# Autodesk Inventor assembly: inner_guide_asm
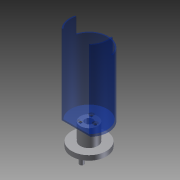
[picture p0: Inventor's stored thumbnail of the model, 180x180]
Saved by Autodesk Inventor 2011 SP2 (Build 150309200, 309)
## iProperties
Created: 2012-05-25
Part Number: inner_guide_asm
Document SubType Name: Assembly
Designer: sungwook
Author: sungwook
## Documents named in this file (3)
- C:\Users\sungwook\Documents\Inventor\Micron20_Base_Tube_Adjst\05222012_Inner_Guide_Tube\inner_guide_asm.iam
- C:\Users\sungwook\Documents\Inventor\Micron20_Base_Tube_Adjst\05222012_Inner_Guide_Tube\ss_inner_guide_top.ipt
- C:\Users\sungwook\Documents\Inventor\Micron20_Base_Tube_Adjst\05222012_Inner_Guide_Tube\ss_inner_guide_bottom.ipt
## Components (2 placed, 2 different names)
1. ss_inner_guide_top:1 — Flush:1, Mate:2, Mate:3, Mate:4
2. ss_inner_guide_bottom:1 — Flush:1, Mate:2, Mate:3, Mate:4
## Relationships (4: Mate 3, Flush 1)
- Flush:1: ss_inner_guide_top:1 ↔ ss_inner_guide_bottom:1
- Mate:2: ss_inner_guide_top:1 ↔ ss_inner_guide_bottom:1
- Mate:3: ss_inner_guide_top:1 ↔ ss_inner_guide_bottom:1
- Mate:4: ss_inner_guide_top:1 ↔ ss_inner_guide_bottom:1
